# Autodesk Inventor assembly: Planter Box
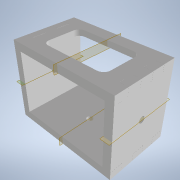
[picture p0: Inventor's stored thumbnail of the model, 180x180]
Saved by Autodesk Inventor 2021.2 (Build 252289000, 289)
## iProperties
Created: 2021-03-04
Part Number: Planter Box
Document SubType Name: Assembly
Designer: 443201246
Author: 443201246
## Documents named in this file (4)
- C:\Users\443201246\Downloads\Planter Box.iam
- C:\Users\443201246\Downloads\Front.ipt
- C:\Users\443201246\Downloads\Side.ipt
- C:\Users\443201246\Downloads\Back.ipt
## Components (4 placed, 2 different names)
1. Front:1 — Flush:1, Flush:2, Flush:3, Mate:1, Flush:4, Flush:5, Flush:6
2. Side:1 — Flush:1, Flush:2, Flush:3, Mate:1, Flush:9
3. Side:2 — Flush:4, Flush:5, Flush:6, Flush:7, Flush:8
4. Front:2 — Flush:7, Flush:8, Flush:9
## Relationships (10: Flush 9, Mate 1)
- Flush:1: Front:1 ↔ Side:1
- Flush:2: Front:1 ↔ Side:1
- Flush:3: Front:1 ↔ Side:1
- Mate:1: Front:1 ↔ Side:1
- Flush:4: Front:1 ↔ Side:2
- Flush:5: Front:1 ↔ Side:2
- Flush:6: Front:1 ↔ Side:2
- Flush:7: Side:2 ↔ Front:2
- Flush:8: Side:2 ↔ Front:2
- Flush:9: Side:1 ↔ Front:2
